# Autodesk Inventor assembly: McCrea_uvodna_snimka_walle
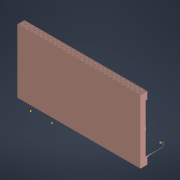
[picture p0: Inventor's stored thumbnail of the model, 180x180]
Saved by Autodesk Inventor 2022 (Build 260153000, 153)
## iProperties
Created: 2022-02-09
Part Number: McCrea_uvodna_snimka_walle
Document SubType Name: Assembly
Designer: MatusBarany
Author: MatusBarany
## Documents named in this file (6)
- C:\Users\MatusBarany\Documents\Inventor\wall-e\assembly\McCrea_uvodna_snimka_walle.iam
- C:\Users\MatusBarany\Documents\Inventor\wall-e\matus\bench\McCrea_assembly_walle.iam
- C:\Users\MatusBarany\Documents\Inventor\wall-e\matus\plocha\McCrea_most_cesta_walle.ipt
- C:\Users\MatusBarany\Documents\Inventor\wall-e\assembly\McCrea_WALLE_bez_HEAD_walle.iam
- C:\Users\MatusBarany\Documents\Inventor\wall-e\matus\lampa\McCrea_lampa_walle.ipt
- C:\Users\MatusBarany\Documents\Inventor\wall-e\lukas\McCrea_Plot_walle.ipt
## Components (8 placed, 5 different names)
1. McCrea_assembly_walle:1 [sub-assembly] — Mate:1, Mate:5
2. McCrea_most_cesta_walle:1 — Mate:1, Mate:2, Mate:3, Mate:4, Mate:6, Mate:7
3. McCrea_WALLE_bez_HEAD_walle:1 [sub-assembly] — Mate:5
4. McCrea_lampa_walle:1 — Mate:2
5. McCrea_lampa_walle:2 — Mate:3
6. McCrea_lampa_walle:3 — Mate:4
7. McCrea_Plot_walle:1 — Mate:6
8. McCrea_Plot_walle:2 — Mate:7
## Relationships (7: Mate 7)
- Mate:1: McCrea_assembly_walle:1 ↔ McCrea_most_cesta_walle:1
- Mate:2: McCrea_most_cesta_walle:1 ↔ McCrea_lampa_walle:1
- Mate:3: McCrea_most_cesta_walle:1 ↔ McCrea_lampa_walle:2
- Mate:4: McCrea_most_cesta_walle:1 ↔ McCrea_lampa_walle:3
- Mate:5: McCrea_assembly_walle:1 ↔ McCrea_WALLE_bez_HEAD_walle:1
- Mate:6: McCrea_most_cesta_walle:1 ↔ McCrea_Plot_walle:1
- Mate:7: McCrea_most_cesta_walle:1 ↔ McCrea_Plot_walle:2
